# Autodesk Inventor assembly: encoder
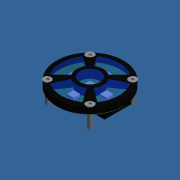
[picture p0: Inventor's stored thumbnail of the model, 180x180]
Saved by Autodesk Inventor 2016 (Build 200138000, 138)
## iProperties
Created: 2015-01-07
Part Number: encoder
Document SubType Name: Assembly
Designer: 4ndreas
Mass: 16.7925 g
Surface Area: 142.599 cm^2
Volume: 12.2137 cm^3
Density: 1.37489 g/cm^3
Author: 4ndreas
## Documents named in this file (5)
- C:\Users\4ndreas\Documents\github\Mantis-Robot-Arm\MantisRobotArm\Workspace\_assemblys\encoder.iam
- C:\Users\4ndreas\Documents\github\Mantis-Robot-Arm\MantisRobotArm\Workspace\_encoder\encoder.ipt
- C:\Users\4ndreas\Documents\github\Mantis-Robot-Arm\MantisRobotArm\Libraries\Content Center Files\de-DE\DIN 7991(2)\DIN 7991 - M3x16.ipt
- C:\Users\4ndreas\Documents\github\Mantis-Robot-Arm\MantisRobotArm\Workspace\_printed parts\encoder_kappe_s.ipt
- C:\Users\4ndreas\Documents\github\Mantis-Robot-Arm\MantisRobotArm\Workspace\_printed parts\encoder_kappe_clear.ipt
## Components (7 placed, 4 different names)
1. encoder:1 — Passend:1, Passend:2, Winkel:1, Passend:10
2. encoder_kappe_s:1 — Passend:1, Passend:2, Passend:4, Passend:5, Passend:6, Passend:7, Passend:8, Fluchtend:4, Passend:9, Passend:10, Passend:11
3. DIN 7991 M3x16:1 — Fluchtend:3, Passend:6
4. DIN 7991 M3x16:2 — Fluchtend:1, Fluchtend:2, Passend:7
5. DIN 7991 M3x16:3 — Fluchtend:2, Fluchtend:3, Passend:8
6. DIN 7991 M3x16:4 — Fluchtend:1, Passend:4, Passend:5
7. encoder_kappe_clear:1 — Fluchtend:4, Passend:9, Passend:11
## Relationships (16: Mate 11, Flush 4, Angle 1)
- Passend:1 [Mate]: encoder:1 ↔ encoder_kappe_s:1
- Passend:2 [Mate]: encoder:1 ↔ encoder_kappe_s:1
- Passend:3 [Mate]
- Winkel:1 [Angle] (90 deg): encoder:1
- Fluchtend:1 [Flush]: DIN 7991 M3x16:2 ↔ DIN 7991 M3x16:4
- Fluchtend:2 [Flush]: DIN 7991 M3x16:2 ↔ DIN 7991 M3x16:3
- Fluchtend:3 [Flush]: DIN 7991 M3x16:1 ↔ DIN 7991 M3x16:3
- Passend:4 [Mate] (-5 mm): encoder_kappe_s:1 ↔ DIN 7991 M3x16:4
- Passend:5 [Mate]: encoder_kappe_s:1 ↔ DIN 7991 M3x16:4
- Passend:6 [Mate]: encoder_kappe_s:1 ↔ DIN 7991 M3x16:1
- Passend:7 [Mate]: encoder_kappe_s:1 ↔ DIN 7991 M3x16:2
- Passend:8 [Mate]: encoder_kappe_s:1 ↔ DIN 7991 M3x16:3
- Fluchtend:4 [Flush] (2 mm): encoder_kappe_s:1 ↔ encoder_kappe_clear:1
- Passend:9 [Mate]: encoder_kappe_s:1 ↔ encoder_kappe_clear:1
- Passend:10 [Mate]: encoder:1 ↔ encoder_kappe_s:1
- Passend:11 [Mate]: encoder_kappe_s:1 ↔ encoder_kappe_clear:1
